# Autodesk Inventor assembly: Trunk
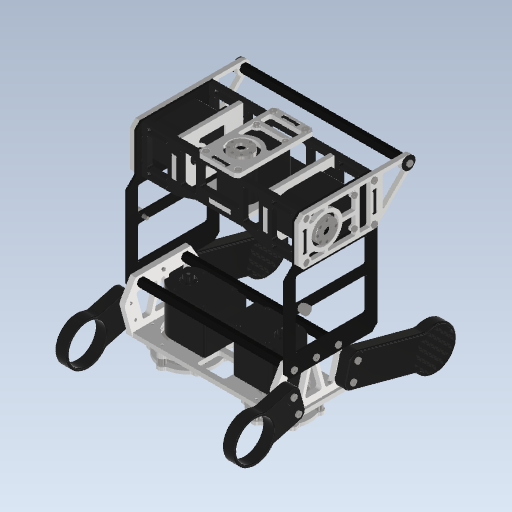
[picture p0: Inventor's stored thumbnail of the model, 512x512]
Saved by Autodesk Inventor 2020.4 (Build 244396000, 396)
## iProperties
Created: 2022-01-05
Part Number: Trunk
Document SubType Name: Assembly
Designer: Masato Kubotera
Mass: 836.462 g
Surface Area: 2738.45 cm^2
Volume: 519.507 cm^3
Density: 1.61011 g/cm^3
Author: Masato Kubotera
## Documents named in this file (26)
- C:\Users\Masato\Documents\Inventor\CIT Brains_Inventor\OpenPlatform_ver3_0 - ver4_1_prototype\UpperBody\Trunk\Trunk.iam
- C:\Users\Masato\Documents\Inventor\CIT Brains_Inventor\OpenPlatform_ver3_0 - ver4_1_prototype\ReadyMade\KONDO\B3M-SC-1040-A.ipt
- C:\Users\Masato\Documents\Inventor\CIT Brains_Inventor\OpenPlatform_ver3_0 - ver4_1_prototype\ReadyMade\KONDO\B3M-SC-1170-A.ipt
- C:\Users\Masato\Documents\Inventor\CIT Brains_Inventor\OpenPlatform_ver3_0 - ver4_1_prototype\UpperBody\Trunk\Trunk_chest_frame.ipt
- C:\Users\Masato\Documents\Inventor\CIT Brains_Inventor\OpenPlatform_ver3_0 - ver4_1_prototype\ReadyMade\InsertNut\IRU-304SW.ipt
- C:\Users\Masato\Documents\Inventor\CIT Brains_Inventor\OpenPlatform_ver3_0 - ver4_1_prototype\UpperBody\Trunk\Trunk_neck_frame.ipt
- C:\Users\Masato\Documents\Inventor\CIT Brains_Inventor\OpenPlatform_ver3_0 - ver4_1_prototype\ReadyMade\Screw\M2_6-15.ipt
- C:\Users\Masato\Documents\Inventor\CIT Brains_Inventor\OpenPlatform_ver3_0 - ver4_1_prototype\ReadyMade\Screw\M3-6.ipt
- C:\Users\Masato\Documents\Inventor\CIT Brains_Inventor\OpenPlatform_ver3_0 - ver4_1_prototype\ReadyMade\Screw\M3-8.ipt
- C:\Users\Masato\Documents\Inventor\CIT Brains_Inventor\OpenPlatform_ver3_0 - ver4_1_prototype\UpperBody\Trunk\Trunk_shoulder_frame.ipt
- C:\Users\Masato\Documents\Inventor\CIT Brains_Inventor\OpenPlatform_ver3_0 - ver4_1_prototype\UpperBody\Trunk\Trunk_upper_side_frame.ipt
- C:\Users\Masato\Documents\Inventor\CIT Brains_Inventor\OpenPlatform_ver3_0 - ver4_1_prototype\ReadyMade\Screw\M3-10.ipt
- C:\Users\Masato\Documents\Inventor\CIT Brains_Inventor\OpenPlatform_ver3_0 - ver4_1_prototype\UpperBody\Trunk\Trunk_shoulder_frame_MIR.ipt
- C:\Users\Masato\Documents\Inventor\CIT Brains_Inventor\OpenPlatform_ver3_0 - ver4_1_prototype\ReadyMade\Washer\UUW-0312-10BH.ipt
- C:\Users\Masato\Documents\Inventor\CIT Brains_Inventor\OpenPlatform_ver3_0 - ver4_1_prototype\UpperBody\Trunk\Trunk_lower_side_frame.ipt
- C:\Users\Masato\Documents\Inventor\CIT Brains_Inventor\OpenPlatform_ver3_0 - ver4_1_prototype\UpperBody\Trunk\Trunk_waisit_frame.ipt
- C:\Users\Masato\Documents\Inventor\CIT Brains_Inventor\OpenPlatform_ver3_0 - ver4_1_prototype\UpperBody\Trunk\CrossRollerBearing\BearingUnit.iam
- C:\Users\Masato\Documents\Inventor\CIT Brains_Inventor\OpenPlatform_ver3_0 - ver4_1_prototype\ReadyMade\KONDO\ClampHorn.ipt
- C:\Users\Masato\Documents\Inventor\CIT Brains_Inventor\OpenPlatform_ver3_0 - ver4_1_prototype\ReadyMade\Screw\620103008.ipt
- C:\Users\Masato\Documents\Inventor\CIT Brains_Inventor\OpenPlatform_ver3_0 - ver4_1_prototype\ReadyMade\Screw\SPNFL-BRN-M3-6.ipt
- C:\Users\Masato\Documents\Inventor\CIT Brains_Inventor\OpenPlatform_ver3_0 - ver4_1_prototype\ReadyMade\Spacer\ABLSBF7-140-M3-N3.ipt
- C:\Users\Masato\Documents\Inventor\CIT Brains_Inventor\OpenPlatform_ver3_0 - ver4_1_prototype\ReadyMade\Spacer\ABLSBF7-157-M3-N3.ipt
- C:\Users\Masato\Documents\Inventor\CIT Brains_Inventor\OpenPlatform_ver3_0 - ver4_1_prototype\ReadyMade\Spacer\BRU-309S.ipt
- C:\Users\Masato\Documents\Inventor\CIT Brains_Inventor\OpenPlatform_ver3_0 - ver4_1_prototype\UpperBody\Trunk\FrontBumper.ipt
- C:\Users\Masato\Documents\Inventor\CIT Brains_Inventor\OpenPlatform_ver3_0 - ver4_1_prototype\UpperBody\Trunk\RearBumper.ipt
- C:\Users\Masato\Documents\Inventor\CIT Brains_Inventor\OpenPlatform_ver3_0 - ver4_1_prototype\UpperBody\Trunk\Trunk_servo_bottom_frame.ipt
## Components (115 placed, 25 different names)
1. B3M-SC-1040-A:1 — 挿入:15, 挿入:16, 挿入:95, 角度:2, 挿入:116, 挿入:198
2. ClampHorn:1 — 挿入:95, 角度:2
3. B3M-SC-1040-A:2 — 挿入:43, 挿入:44, 挿入:96, 角度:3, 挿入:117, 挿入:197
4. ClampHorn:2 — 挿入:96, 角度:3
5. B3M-SC-1040-A:3 — 挿入:63, 挿入:64, 挿入:97, 角度:4, 挿入:118, 挿入:199
6. ClampHorn:3 — 挿入:97, 角度:4
7. B3M-SC-1170-A:1 — 挿入:87, 挿入:88
8. B3M-SC-1170-A:2 — 挿入:89, 挿入:90
9. Trunk_chest_frame:1 — 挿入:2, 挿入:3, 挿入:4, 挿入:6, 挿入:131
10. Trunk_chest_frame:2 — 挿入:7, 挿入:9, 挿入:10, 挿入:11, 挿入:12, 挿入:8
11. Trunk_neck_Upper_frame:1 — 挿入:15, 挿入:16, 挿入:18, 挿入:20, 挿入:25, 挿入:26, 挿入:27, 挿入:28, 挿入:202, 挿入:203
12. Trunk_upper_side_frame:1 — 挿入:29, 挿入:30, 挿入:31, 挿入:32, 挿入:33, 挿入:34, 挿入:35, 挿入:36, 挿入:5, 挿入:119, 挿入:189, 挿入:190, 挿入:193, 挿入:195, 挿入:196
13. Trunk_shoulder_frame:1 — 挿入:33, 挿入:34, 挿入:35, 挿入:36, 挿入:37, 挿入:39, 挿入:38, 挿入:40, 挿入:43, 挿入:44, 挿入:139, 挿入:200, 挿入:201
14. Trunk_upper_side_frame:2 — 挿入:52, 挿入:53, 挿入:54, 挿入:55, 挿入:56, 挿入:57, 挿入:58, 挿入:59, 挿入:120, 挿入:191, 挿入:192, 挿入:194
15. Trunk_shoulder_frame_MIR:1 — 挿入:56, 挿入:57, 挿入:58, 挿入:59, 挿入:63, 挿入:64, 挿入:65, 挿入:66, 挿入:67, 挿入:68, 挿入:71, 挿入:72, 角度:5, 挿入:141
16. UUW-0312-10BH:1 — 挿入:75, 挿入:140
17. UUW-0312-10BH:2 — 挿入:76, 挿入:142
18. Trunk_lower_side_frame:1 — 挿入:145, 挿入:146, 挿入:147, 挿入:148, 挿入:177, 挿入:178, 角度:6, 角度:7, 挿入:179, 挿入:180, 挿入:195, 挿入:196
19. Trunk_lower_side_frame:2 — 挿入:143, 挿入:144, 挿入:149, 挿入:150, 挿入:151, 挿入:152
20. Trunk_waisit_frame:1 — フラッシュ:2, フラッシュ:3, フラッシュ:4, 挿入:83, 挿入:84, 挿入:85, 挿入:86, 挿入:87, 挿入:88, 挿入:89, 挿入:90, 挿入:91, 挿入:92, 挿入:93, 挿入:94, 挿入:121, 挿入:122, 挿入:123, 挿入:124, 挿入:143, 挿入:144, 挿入:177, 挿入:178
21. BearingUnit:1 [sub-assembly] — 挿入:83, 挿入:84
22. BearingUnit:2 [sub-assembly] — 挿入:85, 挿入:86
23. ABLSBF7-140-M3-N3:1 — 角度:6, 挿入:179
24. ABLSBF7-140-M3-N3:2 — 角度:7, 挿入:180
25. ABLSBF7-157-M3-N3:1 — 角度:5, 挿入:139, 挿入:140, 挿入:141, 挿入:142
26. UUW-0312-10BH:3 — 挿入:145, 挿入:153, 挿入:181
27. UUW-0312-10BH:4 — 挿入:146, 挿入:154, 挿入:182
28. UUW-0312-10BH:5 — 挿入:147, 挿入:155, 挿入:185
29. UUW-0312-10BH:6 — 挿入:148, 挿入:156, 挿入:186
30. UUW-0312-10BH:7 — 挿入:149, 挿入:157, 挿入:187
31. UUW-0312-10BH:8 — 挿入:150, 挿入:158, 挿入:188
32. UUW-0312-10BH:9 — 挿入:152, 挿入:160, 挿入:184
33. UUW-0312-10BH:10 — 挿入:151, 挿入:159, 挿入:183
34. BRU-309S:1 — 挿入:153, 挿入:161
35. BRU-309S:2 — 挿入:154, 挿入:162
36. BRU-309S:3 — 挿入:155, 挿入:163
37. BRU-309S:4 — 挿入:156, 挿入:164
38. BRU-309S:5 — 挿入:157, 挿入:165
39. BRU-309S:6 — 挿入:158, 挿入:166
40. BRU-309S:7 — 挿入:159, 挿入:167
41. BRU-309S:8 — 挿入:160, 挿入:168
42. UUW-0312-10BH:11 — 挿入:161, 挿入:169
43. UUW-0312-10BH:12 — 挿入:162, 挿入:170
44. UUW-0312-10BH:13 — 挿入:163, 挿入:171
45. UUW-0312-10BH:14 — 挿入:164, 挿入:172
46. UUW-0312-10BH:15 — 挿入:165, 挿入:173
47. UUW-0312-10BH:16 — 挿入:166, 挿入:174
48. UUW-0312-10BH:17 — 挿入:167, 挿入:175
49. UUW-0312-10BH:18 — 挿入:168, 挿入:176
50. FrontBumper:1 — 挿入:181, 挿入:182
51. FrontBumper:2 — 挿入:183, 挿入:184
52. RearBumper:1 — 挿入:185, 挿入:186
53. RearBumper:2 — 挿入:187, 挿入:188
54. Trunk_servo_bottom_frame:1 — 挿入:198
55. Trunk_servo_bottom_frame:2 — 挿入:197
56. Trunk_servo_bottom_frame:3 — 挿入:199
57. M2_6-15:19 — 挿入:202
58. M2_6-15:20 — 挿入:203
59. M2_6-15:17 — 挿入:201
60. M2_6-15:18 — 挿入:200
61. M3-6:9 — 挿入:169
62. M3-6:10 — 挿入:170
63. M3-6:11 — 挿入:171
64. M3-6:12 — 挿入:172
65. M3-6:13 — 挿入:173
66. M3-6:14 — 挿入:174
67. M3-6:15 — 挿入:176
68. M3-6:16 — 挿入:175
69. M3-10:17 — 挿入:189
70. M3-10:18 — 挿入:190
71. M3-10:19 — 挿入:191
72. M3-10:20 — 挿入:192
73. M3-8:7 — 挿入:193
74. M3-8:8 — 挿入:194
75. M3-10:13 — 挿入:121
76. M3-10:14 — 挿入:122
77. M3-10:15 — 挿入:123
78. M3-10:16 — 挿入:124
79. SPNFL-BRN-M3-6:1 — 挿入:119
80. SPNFL-BRN-M3-6:2 — 挿入:120
81. M3-8:2 — 挿入:28
82. M3-8:1 — 挿入:27
83. M3-6:2 — 挿入:26
84. M3-6:1 — 挿入:25
85. M3-8:4 — 挿入:38
86. M3-8:3 — 挿入:37
87. M3-10:4 — 挿入:40
88. M3-10:3 — 挿入:39
89. M2_6-15:12 — 挿入:72
90. M2_6-15:11 — 挿入:71
91. M3-10:6 — 挿入:68
92. M3-10:5 — 挿入:67
93. M3-8:6 — 挿入:66
94. M3-8:5 — 挿入:65
95. M3-6:4 — 挿入:76
96. M3-6:3 — 挿入:75
97. M2_6-15:16 — 挿入:94
98. M2_6-15:15 — 挿入:93
99. M2_6-15:14 — 挿入:92
100. M2_6-15:13 — 挿入:91
101. 620103008:1 — 挿入:116
102. 620103008:2 — 挿入:117
103. 620103008:3 — 挿入:118
104. IRU-304SW:12 — 挿入:12, 挿入:53
105. IRU-304SW:11 — 挿入:11, 挿入:52
106. IRU-304SW:10 — 挿入:10, 挿入:30
107. IRU-304SW:9 — 挿入:9, 挿入:29
108. IRU-304SW:8 — 挿入:8
109. IRU-304SW:7 — 挿入:7, 挿入:18
110. IRU-304SW:6 — 挿入:6, 挿入:32
111. IRU-304SW:5 — 挿入:5, 挿入:31
112. IRU-304SW:4 — 挿入:4, 挿入:55
113. IRU-304SW:3 — 挿入:3, 挿入:54
114. IRU-304SW:2 — 挿入:2, 挿入:20
115. IRU-304SW:1 — 挿入:131
## Relationships (150: Insert 141, Angle 6, Flush 3)
- 挿入:2 [Insert]: Trunk_chest_frame:1 ↔ IRU-304SW:2
- 挿入:3 [Insert]: Trunk_chest_frame:1 ↔ IRU-304SW:3
- 挿入:4 [Insert]: Trunk_chest_frame:1 ↔ IRU-304SW:4
- 挿入:5 [Insert]: Trunk_upper_side_frame:1 ↔ IRU-304SW:5
- 挿入:6 [Insert]: Trunk_chest_frame:1 ↔ IRU-304SW:6
- 挿入:7 [Insert]: Trunk_chest_frame:2 ↔ IRU-304SW:7
- 挿入:8 [Insert]: Trunk_chest_frame:2 ↔ IRU-304SW:8
- 挿入:9 [Insert]: Trunk_chest_frame:2 ↔ IRU-304SW:9
- 挿入:10 [Insert]: Trunk_chest_frame:2 ↔ IRU-304SW:10
- 挿入:11 [Insert]: Trunk_chest_frame:2 ↔ IRU-304SW:11
- 挿入:12 [Insert]: Trunk_chest_frame:2 ↔ IRU-304SW:12
- 挿入:15 [Insert]: B3M-SC-1040-A:1 ↔ Trunk_neck_Upper_frame:1
- 挿入:16 [Insert]: B3M-SC-1040-A:1 ↔ Trunk_neck_Upper_frame:1
- 挿入:18 [Insert]: Trunk_neck_Upper_frame:1 ↔ IRU-304SW:7
- 挿入:20 [Insert]: Trunk_neck_Upper_frame:1 ↔ IRU-304SW:2
- 挿入:25 [Insert]: Trunk_neck_Upper_frame:1 ↔ M3-6:1
- 挿入:26 [Insert]: Trunk_neck_Upper_frame:1 ↔ M3-6:2
- 挿入:27 [Insert]: Trunk_neck_Upper_frame:1 ↔ M3-8:1
- 挿入:28 [Insert]: Trunk_neck_Upper_frame:1 ↔ M3-8:2
- 挿入:29 [Insert]: Trunk_upper_side_frame:1 ↔ IRU-304SW:9
- 挿入:30 [Insert]: Trunk_upper_side_frame:1 ↔ IRU-304SW:10
- 挿入:31 [Insert]: Trunk_upper_side_frame:1 ↔ IRU-304SW:5
- 挿入:32 [Insert]: Trunk_upper_side_frame:1 ↔ IRU-304SW:6
- 挿入:33 [Insert]: Trunk_upper_side_frame:1 ↔ Trunk_shoulder_frame:1
- 挿入:34 [Insert]: Trunk_upper_side_frame:1 ↔ Trunk_shoulder_frame:1
- 挿入:35 [Insert]: Trunk_upper_side_frame:1 ↔ Trunk_shoulder_frame:1
- 挿入:36 [Insert]: Trunk_upper_side_frame:1 ↔ Trunk_shoulder_frame:1
- 挿入:37 [Insert]: Trunk_shoulder_frame:1 ↔ M3-8:3
- 挿入:39 [Insert]: Trunk_shoulder_frame:1 ↔ M3-10:3
- 挿入:38 [Insert]: Trunk_shoulder_frame:1 ↔ M3-8:4
- 挿入:40 [Insert]: Trunk_shoulder_frame:1 ↔ M3-10:4
- 挿入:43 [Insert]: B3M-SC-1040-A:2 ↔ Trunk_shoulder_frame:1
- 挿入:44 [Insert]: B3M-SC-1040-A:2 ↔ Trunk_shoulder_frame:1
- 挿入:52 [Insert]: Trunk_upper_side_frame:2 ↔ IRU-304SW:11
- 挿入:53 [Insert]: Trunk_upper_side_frame:2 ↔ IRU-304SW:12
- 挿入:54 [Insert]: Trunk_upper_side_frame:2 ↔ IRU-304SW:3
- 挿入:55 [Insert]: Trunk_upper_side_frame:2 ↔ IRU-304SW:4
- 挿入:56 [Insert]: Trunk_upper_side_frame:2 ↔ Trunk_shoulder_frame_MIR:1
- 挿入:57 [Insert]: Trunk_upper_side_frame:2 ↔ Trunk_shoulder_frame_MIR:1
- 挿入:58 [Insert]: Trunk_upper_side_frame:2 ↔ Trunk_shoulder_frame_MIR:1
- 挿入:59 [Insert]: Trunk_upper_side_frame:2 ↔ Trunk_shoulder_frame_MIR:1
- 挿入:63 [Insert]: B3M-SC-1040-A:3 ↔ Trunk_shoulder_frame_MIR:1
- 挿入:64 [Insert]: B3M-SC-1040-A:3 ↔ Trunk_shoulder_frame_MIR:1
- 挿入:65 [Insert]: Trunk_shoulder_frame_MIR:1 ↔ M3-8:5
- 挿入:66 [Insert]: Trunk_shoulder_frame_MIR:1 ↔ M3-8:6
- 挿入:67 [Insert]: Trunk_shoulder_frame_MIR:1 ↔ M3-10:5
- 挿入:68 [Insert]: Trunk_shoulder_frame_MIR:1 ↔ M3-10:6
- 挿入:71 [Insert]: Trunk_shoulder_frame_MIR:1 ↔ M2_6-15:11
- 挿入:72 [Insert]: Trunk_shoulder_frame_MIR:1 ↔ M2_6-15:12
- 挿入:75 [Insert]: UUW-0312-10BH:1 ↔ M3-6:3
- 挿入:76 [Insert]: UUW-0312-10BH:2 ↔ M3-6:4
- フラッシュ:2 [Flush]: Trunk_waisit_frame:1
- フラッシュ:3 [Flush]: Trunk_waisit_frame:1
- フラッシュ:4 [Flush]: Trunk_waisit_frame:1
- 挿入:83 [Insert]: Trunk_waisit_frame:1 ↔ BearingUnit:1
- 挿入:84 [Insert]: Trunk_waisit_frame:1 ↔ BearingUnit:1
- 挿入:85 [Insert]: Trunk_waisit_frame:1 ↔ BearingUnit:2
- 挿入:86 [Insert]: Trunk_waisit_frame:1 ↔ BearingUnit:2
- 挿入:87 [Insert]: B3M-SC-1170-A:1 ↔ Trunk_waisit_frame:1
- 挿入:88 [Insert]: B3M-SC-1170-A:1 ↔ Trunk_waisit_frame:1
- 挿入:89 [Insert]: B3M-SC-1170-A:2 ↔ Trunk_waisit_frame:1
- 挿入:90 [Insert]: B3M-SC-1170-A:2 ↔ Trunk_waisit_frame:1
- 挿入:91 [Insert]: Trunk_waisit_frame:1 ↔ M2_6-15:13
- 挿入:92 [Insert]: Trunk_waisit_frame:1 ↔ M2_6-15:14
- 挿入:93 [Insert]: Trunk_waisit_frame:1 ↔ M2_6-15:15
- 挿入:94 [Insert]: Trunk_waisit_frame:1 ↔ M2_6-15:16
- 挿入:95 [Insert]: B3M-SC-1040-A:1 ↔ ClampHorn:1
- 挿入:96 [Insert]: B3M-SC-1040-A:2 ↔ ClampHorn:2
- 挿入:97 [Insert]: B3M-SC-1040-A:3 ↔ ClampHorn:3
- 角度:2 [Angle] (0 deg): B3M-SC-1040-A:1 ↔ ClampHorn:1
- 角度:3 [Angle] (0 deg): B3M-SC-1040-A:2 ↔ ClampHorn:2
- 角度:4 [Angle] (0 deg): B3M-SC-1040-A:3 ↔ ClampHorn:3
- 挿入:116 [Insert]: B3M-SC-1040-A:1 ↔ 620103008:1
- 挿入:117 [Insert]: B3M-SC-1040-A:2 ↔ 620103008:2
- 挿入:118 [Insert]: B3M-SC-1040-A:3 ↔ 620103008:3
- 挿入:119 [Insert]: Trunk_upper_side_frame:1 ↔ SPNFL-BRN-M3-6:1
- 挿入:120 [Insert]: Trunk_upper_side_frame:2 ↔ SPNFL-BRN-M3-6:2
- 挿入:121 [Insert]: Trunk_waisit_frame:1 ↔ M3-10:13
- 挿入:122 [Insert]: Trunk_waisit_frame:1 ↔ M3-10:14
- 挿入:123 [Insert]: Trunk_waisit_frame:1 ↔ M3-10:15
- 挿入:124 [Insert]: Trunk_waisit_frame:1 ↔ M3-10:16
- 挿入:131 [Insert]: Trunk_chest_frame:1 ↔ IRU-304SW:1
- 角度:5 [Angle] (0 deg): Trunk_shoulder_frame_MIR:1 ↔ ABLSBF7-157-M3-N3:1
- 挿入:139 [Insert]: Trunk_shoulder_frame:1 ↔ ABLSBF7-157-M3-N3:1
- 挿入:140 [Insert]: UUW-0312-10BH:1 ↔ ABLSBF7-157-M3-N3:1
- 挿入:141 [Insert]: Trunk_shoulder_frame_MIR:1 ↔ ABLSBF7-157-M3-N3:1
- 挿入:142 [Insert]: UUW-0312-10BH:2 ↔ ABLSBF7-157-M3-N3:1
- 挿入:143 [Insert]: Trunk_lower_side_frame:2 ↔ Trunk_waisit_frame:1
- 挿入:144 [Insert]: Trunk_lower_side_frame:2 ↔ Trunk_waisit_frame:1
- 挿入:145 [Insert]: Trunk_lower_side_frame:1 ↔ UUW-0312-10BH:3
- 挿入:146 [Insert]: Trunk_lower_side_frame:1 ↔ UUW-0312-10BH:4
- 挿入:147 [Insert]: Trunk_lower_side_frame:1 ↔ UUW-0312-10BH:5
- 挿入:148 [Insert]: Trunk_lower_side_frame:1 ↔ UUW-0312-10BH:6
- 挿入:149 [Insert]: Trunk_lower_side_frame:2 ↔ UUW-0312-10BH:7
- 挿入:150 [Insert]: Trunk_lower_side_frame:2 ↔ UUW-0312-10BH:8
- 挿入:151 [Insert]: Trunk_lower_side_frame:2 ↔ UUW-0312-10BH:10
- 挿入:152 [Insert]: Trunk_lower_side_frame:2 ↔ UUW-0312-10BH:9
- 挿入:153 [Insert]: UUW-0312-10BH:3 ↔ BRU-309S:1
- 挿入:154 [Insert]: UUW-0312-10BH:4 ↔ BRU-309S:2
- 挿入:155 [Insert]: UUW-0312-10BH:5 ↔ BRU-309S:3
- 挿入:156 [Insert]: UUW-0312-10BH:6 ↔ BRU-309S:4
- 挿入:157 [Insert]: UUW-0312-10BH:7 ↔ BRU-309S:5
- 挿入:158 [Insert]: UUW-0312-10BH:8 ↔ BRU-309S:6
- 挿入:159 [Insert]: UUW-0312-10BH:10 ↔ BRU-309S:7
- 挿入:160 [Insert]: UUW-0312-10BH:9 ↔ BRU-309S:8
- 挿入:161 [Insert]: BRU-309S:1 ↔ UUW-0312-10BH:11
- 挿入:162 [Insert]: BRU-309S:2 ↔ UUW-0312-10BH:12
- 挿入:163 [Insert]: BRU-309S:3 ↔ UUW-0312-10BH:13
- 挿入:164 [Insert]: BRU-309S:4 ↔ UUW-0312-10BH:14
- 挿入:165 [Insert]: BRU-309S:5 ↔ UUW-0312-10BH:15
- 挿入:166 [Insert]: BRU-309S:6 ↔ UUW-0312-10BH:16
- 挿入:167 [Insert]: BRU-309S:7 ↔ UUW-0312-10BH:17
- 挿入:168 [Insert]: BRU-309S:8 ↔ UUW-0312-10BH:18
- 挿入:169 [Insert]: UUW-0312-10BH:11 ↔ M3-6:9
- 挿入:170 [Insert]: UUW-0312-10BH:12 ↔ M3-6:10
- 挿入:171 [Insert]: UUW-0312-10BH:13 ↔ M3-6:11
- 挿入:172 [Insert]: UUW-0312-10BH:14 ↔ M3-6:12
- 挿入:173 [Insert]: UUW-0312-10BH:15 ↔ M3-6:13
- 挿入:174 [Insert]: UUW-0312-10BH:16 ↔ M3-6:14
- 挿入:175 [Insert]: UUW-0312-10BH:17 ↔ M3-6:16
- 挿入:176 [Insert]: UUW-0312-10BH:18 ↔ M3-6:15
- 挿入:177 [Insert]: Trunk_lower_side_frame:1 ↔ Trunk_waisit_frame:1
- 挿入:178 [Insert]: Trunk_lower_side_frame:1 ↔ Trunk_waisit_frame:1
- 角度:6 [Angle] (0 deg): Trunk_lower_side_frame:1 ↔ ABLSBF7-140-M3-N3:1
- 角度:7 [Angle] (0 deg): Trunk_lower_side_frame:1 ↔ ABLSBF7-140-M3-N3:2
- 挿入:179 [Insert]: Trunk_lower_side_frame:1 ↔ ABLSBF7-140-M3-N3:1
- 挿入:180 [Insert]: Trunk_lower_side_frame:1 ↔ ABLSBF7-140-M3-N3:2
- 挿入:181 [Insert]: UUW-0312-10BH:3 ↔ FrontBumper:1
- 挿入:182 [Insert]: UUW-0312-10BH:4 ↔ FrontBumper:1
- 挿入:183 [Insert]: UUW-0312-10BH:10 ↔ FrontBumper:2
- 挿入:184 [Insert]: UUW-0312-10BH:9 ↔ FrontBumper:2
- 挿入:185 [Insert]: UUW-0312-10BH:5 ↔ RearBumper:1
- 挿入:186 [Insert]: UUW-0312-10BH:6 ↔ RearBumper:1
- 挿入:187 [Insert]: UUW-0312-10BH:7 ↔ RearBumper:2
- 挿入:188 [Insert]: UUW-0312-10BH:8 ↔ RearBumper:2
- 挿入:189 [Insert]: Trunk_upper_side_frame:1 ↔ M3-10:17
- 挿入:190 [Insert]: Trunk_upper_side_frame:1 ↔ M3-10:18
- 挿入:191 [Insert]: Trunk_upper_side_frame:2 ↔ M3-10:19
- 挿入:192 [Insert]: Trunk_upper_side_frame:2 ↔ M3-10:20
- 挿入:193 [Insert]: Trunk_upper_side_frame:1 ↔ M3-8:7
- 挿入:194 [Insert]: Trunk_upper_side_frame:2 ↔ M3-8:8
- 挿入:195 [Insert]: Trunk_upper_side_frame:1 ↔ Trunk_lower_side_frame:1
- 挿入:196 [Insert]: Trunk_upper_side_frame:1 ↔ Trunk_lower_side_frame:1
- 挿入:197 [Insert]: B3M-SC-1040-A:2 ↔ Trunk_servo_bottom_frame:2
- 挿入:198 [Insert]: B3M-SC-1040-A:1 ↔ Trunk_servo_bottom_frame:1
- 挿入:199 [Insert]: B3M-SC-1040-A:3 ↔ Trunk_servo_bottom_frame:3
- 挿入:200 [Insert]: Trunk_shoulder_frame:1 ↔ M2_6-15:18
- 挿入:201 [Insert]: Trunk_shoulder_frame:1 ↔ M2_6-15:17
- 挿入:202 [Insert]: Trunk_neck_Upper_frame:1 ↔ M2_6-15:19
- 挿入:203 [Insert]: Trunk_neck_Upper_frame:1 ↔ M2_6-15:20
